# Autodesk Inventor assembly: ASY GBK 1210 long wall shield 3
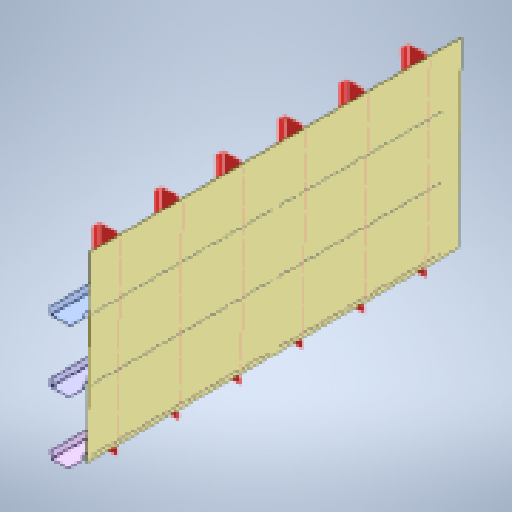
[picture p0: Inventor's stored thumbnail of the model, 512x512]
Saved by Autodesk Inventor 2026 (Build 300175000, 175)
## iProperties
Created: 2026-05-07
Part Number: ASY GBK 1210 long wall shield 3
Document SubType Name: Assembly
Designer: pokla
Mass: 252568 g
Surface Area: 163192 cm^2
Volume: 32174.3 cm^3
Density: 7.85 g/cm^3
Stock Number: 1211
Author: admin
## Documents named in this file (7)
- C:\Users\pokla\Documents\Inventor\GBK-Gubkinskiy\ASY GBK 1210 long wall shield 3.iam
- C:\Users\pokla\Documents\Inventor\GBK-Gubkinskiy\GBK 1211 shield 2.ipt
- C:\Users\pokla\Documents\Inventor\GBK-Gubkinskiy\GBK 0201 second rib.ipt
- C:\Users\pokla\Documents\Inventor\GBK-Gubkinskiy\GBK 0202 stringer 4.ipt
- C:\Users\pokla\Documents\Inventor\GBK-Gubkinskiy\GBK 0203 stringer 5.ipt
- C:\Users\pokla\Documents\Inventor\GBK-Gubkinskiy\GBK 0204 stringer 6.ipt
- C:\Users\pokla\Documents\Inventor\GBK-Gubkinskiy\GBK 0101 main rib.ipt
## Components (13 placed, 6 different names)
1. GBK 0202 stringer 4.ipt:1
2. GBK 0202 stringer 4.ipt:2
3. GBK 0203 stringer 5.ipt:1
4. GBK 0203 stringer 5.ipt:2
5. GBK 0204 stringer 6.ipt:1
6. GBK 0204 stringer 6.ipt:2
7. GBK 1211 shield 2.ipt:1
8. GBK 0201 second rib.ipt:1
9. 04.2 GBK rib:2
10. 04.2 GBK rib:3
11. 04.2 GBK rib:4
12. 04.2 GBK rib:5
13. 04.2 GBK rib:6
## Component patterns: (6 elements, first: GBK 0201 second rib.ipt:1)
## Relationships (9: WeldJoint 6, Mate 2, Flush 1)
- [Flush] (250 mm): GBK 1211 shield 2.ipt:1 ↔ GBK 0201 second rib.ipt:1
- [Mate]: GBK 1211 shield 2.ipt:1 ↔ GBK 0201 second rib.ipt:1
- [Mate]: GBK 1211 shield 2.ipt:1 ↔ GBK 0201 second rib.ipt:1
- [WeldJoint]: GBK 0202 stringer 4.ipt:1 ↔ GBK 0202 stringer 4.ipt:2
- [WeldJoint]: GBK 0203 stringer 5.ipt:1 ↔ GBK 0203 stringer 5.ipt:2
- [WeldJoint]: GBK 0204 stringer 6.ipt:1 ↔ GBK 0204 stringer 6.ipt:2
- [WeldJoint] (4 mm): GBK 0204 stringer 6.ipt:1 ↔ GBK 0201 second rib.ipt:1
- [WeldJoint] (4 mm): GBK 0203 stringer 5.ipt:1 ↔ GBK 0201 second rib.ipt:1
- [WeldJoint] (4 mm): GBK 0202 stringer 4.ipt:1 ↔ GBK 0201 second rib.ipt:1
## Named parameters: Шаг_шпангоутов = 496.66667 mm
